# Autodesk Inventor assembly: CLB_074_PulleyAssembly
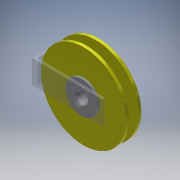
[picture p0: Inventor's stored thumbnail of the model, 180x180]
Saved by Autodesk Inventor 2018.3 (Build 223284000, 284)
## iProperties
Created: 2020-02-17
Part Number: CLB_074_PulleyAssembly
Document SubType Name: Assembly
Designer: 22perngrac
Author: 22perngrac
## Documents named in this file (4)
- C:\Users\22perngrac\Documents\GrabCAD\Infinite Recharge 2020\Build season\CLB_074_PulleyAssembly.iam
- C:\Users\22perngrac\Documents\GrabCAD\Infinite Recharge 2020\Build season\CLB_073_BallBearing.ipt
- C:\Users\22perngrac\Documents\GrabCAD\Infinite Recharge 2020\Build season\CLB_072_ScissorPulley.ipt
- C:\Users\22perngrac\Documents\GrabCAD\Infinite Recharge 2020\Build season\CLB_081_ScissorRopeKeeper.ipt
## Components (4 placed, 3 different names)
1. CLB_073_BallBearing:1 — Insert:1, Mate:1, Mate:2
2. CLB_073_BallBearing:2 — Insert:2
3. CLB_072_ScissorPulley:1 — Insert:1, Insert:2
4. CLB_081_ScissorRopeKeeper:1 — Mate:1, Mate:2
## Relationships (4: Insert 2, Mate 2)
- Insert:1: CLB_073_BallBearing:1 ↔ CLB_072_ScissorPulley:1
- Insert:2: CLB_073_BallBearing:2 ↔ CLB_072_ScissorPulley:1
- Mate:1: CLB_073_BallBearing:1 ↔ CLB_081_ScissorRopeKeeper:1
- Mate:2: CLB_073_BallBearing:1 ↔ CLB_081_ScissorRopeKeeper:1
